# Autodesk Inventor assembly: recovery_structure2_asm
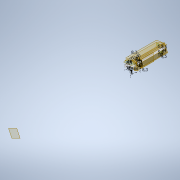
[picture p0: Inventor's stored thumbnail of the model, 180x180]
Saved by Autodesk Inventor 2020 (Build 240168000, 168)
## iProperties
Created: 2022-05-20
Part Number: recovery_structure2_asm
Document SubType Name: Assembly
Designer: sp
Author: sp
## Documents named in this file (7)
- C:\Users\sp\Documents\Rocket\rocket\CAD\recovery_structure2_asm.iam
- C:\Users\sp\Documents\Rocket\rocket\CAD\Verbindungsring_top.ipt
- C:\Users\sp\Documents\Rocket\rocket\CAD\Verbindungsring_bottom.ipt
- C:\Users\sp\Documents\Rocket\rocket\CAD\stange2.ipt
- C:\Users\sp\Documents\Rocket\rocket\CAD\Deckel_Parachute_6.ipt
- C:\Users\sp\Documents\Rocket\rocket\CAD\Deckel_Parachute_5.ipt
- C:\Users\sp\Documents\Rocket\rocket\CAD\Servo_Kupplung_V2.ipt
## Components (7 placed, 6 different names)
1. Verbindungsring_top:1 — Einfügen:1, Einfügen:2, Einfügen:5
2. Verbindungsring_bottom:1 — Einfügen:3, Passend:1
3. stange2:1 — Einfügen:1, Passend:1, Passend:2
4. stange2:2 — Einfügen:2, Einfügen:3, Passend:3
5. Deckel_Parachute_6:1 — Passend:2, Passend:3, Einfügen:6
6. Deckel_Parachute_5:1 — Einfügen:6
7. Servo_Kupplung_V2:1 — Einfügen:5
## Relationships (8: Insert 5, Mate 3)
- Einfügen:1 [Insert]: Verbindungsring_top:1 ↔ stange2:1
- Einfügen:2 [Insert]: Verbindungsring_top:1 ↔ stange2:2
- Einfügen:3 [Insert]: Verbindungsring_bottom:1 ↔ stange2:2
- Passend:1 [Mate]: Verbindungsring_bottom:1 ↔ stange2:1
- Passend:2 [Mate]: stange2:1 ↔ Deckel_Parachute_6:1
- Passend:3 [Mate]: stange2:2 ↔ Deckel_Parachute_6:1
- Einfügen:5 [Insert] (-5 mm): Verbindungsring_top:1 ↔ Servo_Kupplung_V2:1
- Einfügen:6 [Insert] (1 mm): Deckel_Parachute_6:1 ↔ Deckel_Parachute_5:1
